# Autodesk Inventor assembly: tapa1
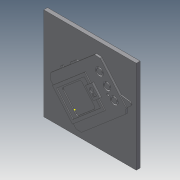
[picture p0: Inventor's stored thumbnail of the model, 180x180]
Saved by Autodesk Inventor 2017 (Build 210142000, 142)
## iProperties
Created: 2020-06-12
Part Number: tapa1
Document SubType Name: Assembly
Designer: c
Author: c
## Documents named in this file (3)
- C:\Users\c\Desktop\dcom\tapa1.iam
- C:\Users\c\Desktop\dcom\dibujo.ipt
- C:\Users\c\Desktop\dcom\tapa.ipt
## Components (2 placed, 2 different names)
1. dibujo:1 — Mate:1
2. tapa:1 — Mate:1
## Relationships (1: Mate 1)
- Mate:1: dibujo:1 ↔ tapa:1
